# Autodesk Inventor assembly: ND Motor Left
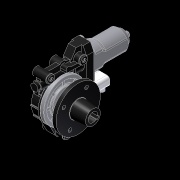
[picture p0: Inventor's stored thumbnail of the model, 180x180]
Saved by Autodesk Inventor 2012 (Build 160160000, 160)
## iProperties
Company: Team 801
Shininess: 64.0
Length Units: 11272
Angle Units: 11279
Time Units: 11290
Mass Units: 11286
Length Display Precision: 3
Angle Display Precision: 2
Compacted: True
Part Number: ND Motor Left
Document SubType Name: Assembly
Created: 2006-02-01
Designer: Jeffrey M
Catalog Web Link: www.team801.org
Density: 0.0
Volumn: 0.0
Area: 0.0
PropertySet Name: Model Information
Control State: 0
Master: False
Checked Out: False
Author: Jeffrey M
## Documents named in this file (3)
- Z:\UserData\Documents\Inventor\team1885frc\KOP Motors\ND Motor Left.iam
- Z:\UserData\Documents\Inventor\team1885frc\KOP Motors\ND Motor Left.ipt
- Z:\UserData\Documents\Inventor\team1885frc\KOP Motors\nippondensogearcoupler2.ipt
## Components (2 placed, 2 different names)
1. ND Motor Left:1 — Mate:1, Angle:1, Mate:2
2. nippondensogearcoupler2:1 — Mate:1, Angle:1, Mate:2
## Relationships (3: Mate 2, Angle 1)
- Mate:1: ND Motor Left:1 ↔ nippondensogearcoupler2:1
- Angle:1 (0 deg): ND Motor Left:1 ↔ nippondensogearcoupler2:1
- Mate:2: ND Motor Left:1 ↔ nippondensogearcoupler2:1
